# Autodesk Inventor assembly: Stewart-Platform-Innen
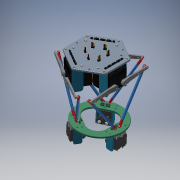
[picture p0: Inventor's stored thumbnail of the model, 180x180]
Saved by Autodesk Inventor 2018.2 (Build 222227000, 227)
## iProperties
Created: 2018-02-17
Part Number: Stewart-Platform-Innen
Material: Generisch
Document SubType Name: Assembly
Designer: JochenAlt
Author: JochenAlt
## Documents named in this file (11)
- D:\Projects\Donna\CAD\Stewart-Platform-Inside.iam
- D:\Projects\Donna\CAD\Servo-Holder.iam
- D:\Projects\Donna\CAD\Stewart-Platform-Base-Inside.ipt
- D:\Projects\Donna\CAD\Ball-Joint-Rod.iam
- D:\Projects\Donna\CAD\Servo-Arm-52mm-Ball-Joint.iam
- D:\Projects\Donna\CAD\Stewart-Plate-Inside.iam
- C:\Users\JochenAlt\Documents\Inventor\Content Center Files\R2018\de-DE\DIN 912\DIN 912 - M2 x 0,4 x 6 x 5.ipt
- C:\Users\JochenAlt\Documents\Inventor\Content Center Files\R2018\de-DE\AS 1112 (2)\AS 1112 - M2  Typ 5.ipt
- C:\Users\JochenAlt\Documents\Inventor\Content Center Files\R2018\de-DE\DIN 912\DIN 912 - M3 x 0,5 x 12 x 10,75.ipt
- C:\Users\JochenAlt\Documents\Inventor\Content Center Files\R2018\de-DE\DIN 912\DIN 912 - M3 x 0,5 x 10 x 8,75.ipt
- C:\Users\JochenAlt\Documents\Inventor\Content Center Files\R2018\de-DE\AS 1112 (2)\AS 1112 - M3  Typ 5.ipt
## Components (69 placed, 10 different names)
1. ServoHolder:1 [sub-assembly] — Passend:3, Passend:4, Passend:31, Passend:32, Passend:33, Passend:34, Passend:35, Passend:36, Passend:37, Passend:38, Passend:79, Passend:80, Passend:81, Passend:82, Passend:102, Passend:104, Passend:106, Passend:108, Passend:118, Passend:121, Passend:122, Passend:123, Passend:131, Passend:133
2. ServoHolder:2 [sub-assembly] — Passend:5, Passend:6, Einfügen:1, Einfügen:2, Einfügen:3, Einfügen:4, Passend:83, Passend:84, Passend:85, Passend:86, Passend:88, Passend:90, Passend:92, Passend:94, Passend:119, Passend:120, Passend:126, Passend:127, Passend:135
3. ServoHolder:3 [sub-assembly] — Passend:1, Passend:2, Passend:39, Passend:40, Passend:41, Passend:42, Passend:43, Passend:44, Passend:45, Passend:46, Passend:75, Passend:76, Passend:77, Passend:78, Passend:96, Einfügen:5, Passend:98, Passend:100, Passend:116, Passend:117, Passend:124, Passend:125, Passend:137, Passend:139
4. Stewart-Platform-Base:1 — Passend:1, Passend:2, Passend:3, Passend:4, Passend:5, Passend:6, Passend:48, Passend:50, Passend:52, Passend:54, Passend:56, Passend:58, Passend:60, Passend:62, Passend:64, Passend:66, Passend:68, Passend:70, Passend:71, Passend:72, Passend:73, Passend:74, Passend:128, Passend:129
5. Ball Joint Rod:1 [sub-assembly] — Passend:12, Passend:113
6. Ball Joint Rod:2 [sub-assembly] — Passend:9, Passend:115
7. Servo Lever ball joint:1 [sub-assembly] — Passend:12, Passend:121, Passend:122
8. Servo Lever ball joint:2 [sub-assembly] — Passend:9, Passend:118, Passend:123
9. Servo Lever ball joint:3 [sub-assembly] — Passend:18, Passend:117, Passend:125
10. Servo Lever ball joint:4 [sub-assembly] — Passend:17, Passend:116, Passend:124
11. Servo Lever ball joint:5 [sub-assembly] — Passend:24, Passend:119, Passend:127
12. Servo Lever ball joint:6 [sub-assembly] — Passend:23, Passend:120, Passend:126
13. Ball Joint Rod:3 [sub-assembly] — Passend:17, Passend:109
14. Ball Joint Rod:4 [sub-assembly] — Passend:18, Passend:110
15. Ball Joint Rod:5 [sub-assembly] — Passend:24, Passend:111
16. Ball Joint Rod:6 [sub-assembly] — Passend:23, Passend:114
17. DIN 912 - ersetzt durch DIN EN ISO 4762 M2 x 6:1 — Einfügen:1, Passend:53
18. DIN 912 - ersetzt durch DIN EN ISO 4762 M2 x 6:2 — Einfügen:2, Passend:47
19. DIN 912 - ersetzt durch DIN EN ISO 4762 M2 x 6:3 — Einfügen:3, Passend:49
20. DIN 912 - ersetzt durch DIN EN ISO 4762 M2 x 6:4 — Einfügen:4, Passend:51
21. DIN 912 - ersetzt durch DIN EN ISO 4762 M2 x 6:5 — Passend:31, Passend:32, Passend:67
22. DIN 912 - ersetzt durch DIN EN ISO 4762 M2 x 6:6 — Passend:33, Passend:34, Passend:63
23. DIN 912 - ersetzt durch DIN EN ISO 4762 M2 x 6:7 — Passend:35, Passend:36, Passend:65
24. DIN 912 - ersetzt durch DIN EN ISO 4762 M2 x 6:8 — Passend:37, Passend:38, Passend:69
25. DIN 912 - ersetzt durch DIN EN ISO 4762 M2 x 6:9 — Passend:39, Passend:40, Passend:55
26. DIN 912 - ersetzt durch DIN EN ISO 4762 M2 x 6:10 — Passend:41, Passend:42, Passend:57
27. DIN 912 - ersetzt durch DIN EN ISO 4762 M2 x 6:11 — Passend:43, Passend:44, Passend:59
28. DIN 912 - ersetzt durch DIN EN ISO 4762 M2 x 6:12 — Passend:45, Passend:46, Passend:61
29. AS 1112 (2) - Metrisch M2  Typ 5:1 — Passend:47, Passend:48
30. AS 1112 (2) - Metrisch M2  Typ 5:2 — Passend:49, Passend:50
31. AS 1112 (2) - Metrisch M2  Typ 5:3 — Passend:51, Passend:52
32. AS 1112 (2) - Metrisch M2  Typ 5:4 — Passend:53, Passend:54
33. AS 1112 (2) - Metrisch M2  Typ 5:5 — Passend:55, Passend:56
34. AS 1112 (2) - Metrisch M2  Typ 5:6 — Passend:57, Passend:58
35. AS 1112 (2) - Metrisch M2  Typ 5:7 — Passend:59, Passend:60
36. AS 1112 (2) - Metrisch M2  Typ 5:8 — Passend:61, Passend:62
37. AS 1112 (2) - Metrisch M2  Typ 5:9 — Passend:63, Passend:64
38. AS 1112 (2) - Metrisch M2  Typ 5:10 — Passend:65, Passend:66
39. AS 1112 (2) - Metrisch M2  Typ 5:11 — Passend:67, Passend:68
40. AS 1112 (2) - Metrisch M2  Typ 5:12 — Passend:69, Passend:70
41. DIN 912 - ersetzt durch DIN EN ISO 4762 M3 x 12:4 — Passend:73, Passend:74, Passend:138
42. DIN 912 - ersetzt durch DIN EN ISO 4762 M3 x 10:1 — Passend:75, Passend:76, Passend:97
43. DIN 912 - ersetzt durch DIN EN ISO 4762 M3 x 10:2 — Passend:77, Passend:78, Passend:99
44. DIN 912 - ersetzt durch DIN EN ISO 4762 M3 x 10:3 — Passend:79, Passend:80, Passend:101
45. DIN 912 - ersetzt durch DIN EN ISO 4762 M3 x 10:4 — Passend:81, Passend:82, Passend:107
46. DIN 912 - ersetzt durch DIN EN ISO 4762 M3 x 10:5 — Passend:83, Passend:84, Passend:89
47. DIN 912 - ersetzt durch DIN EN ISO 4762 M3 x 10:6 — Passend:85, Passend:86, Passend:93
48. AS 1112 (2) - Metrisch M3  Typ 5:1 — Passend:87, Passend:88
49. AS 1112 (2) - Metrisch M3  Typ 5:2 — Passend:89, Passend:90
50. AS 1112 (2) - Metrisch M3  Typ 5:3 — Passend:92
51. AS 1112 (2) - Metrisch M3  Typ 5:4 — Passend:93, Passend:94
52. AS 1112 (2) - Metrisch M3  Typ 5:5 — Passend:95, Passend:96
53. AS 1112 (2) - Metrisch M3  Typ 5:6 — Einfügen:5
54. AS 1112 (2) - Metrisch M3  Typ 5:7 — Passend:97, Passend:98
55. AS 1112 (2) - Metrisch M3  Typ 5:8 — Passend:99, Passend:100
56. AS 1112 (2) - Metrisch M3  Typ 5:9 — Passend:101, Passend:102
57. AS 1112 (2) - Metrisch M3  Typ 5:10 — Passend:104
58. AS 1112 (2) - Metrisch M3  Typ 5:11 — Passend:105, Passend:106
59. AS 1112 (2) - Metrisch M3  Typ 5:12 — Passend:107, Passend:108
60. Stewart-Plate:1 [sub-assembly] — Passend:109, Passend:110, Passend:111, Passend:113, Passend:114, Passend:115
61. DIN 912 - ersetzt durch DIN EN ISO 4762 M3 x 12:5 — Passend:128, Passend:129, Passend:130
62. AS 1112 (2) - Metrisch M3  Typ 5:13 — Passend:130, Passend:131
63. AS 1112 (2) - Metrisch M3  Typ 5:14 — Passend:132, Passend:133
64. AS 1112 (2) - Metrisch M3  Typ 5:15 — Passend:134, Passend:135
65. AS 1112 (2) - Metrisch M3  Typ 5:16 — Passend:136, Passend:137
66. AS 1112 (2) - Metrisch M3  Typ 5:17 — Passend:138, Passend:139
67. DIN 912 - ersetzt durch DIN EN ISO 4762 M3 x 12:1 — Passend:71, Passend:72, Passend:95, Passend:136
68. DIN 912 - ersetzt durch DIN EN ISO 4762 M3 x 12:2 — Passend:105, Passend:132
69. DIN 912 - ersetzt durch DIN EN ISO 4762 M3 x 12:3 — Passend:87, Passend:134
## Component patterns: (3 elements, first: DIN 912 - ersetzt durch DIN EN ISO 4762 M3 x 12:1)
## Relationships (123: Mate 118, Insert 5)
- Passend:1 [Mate]: ServoHolder:3 ↔ Stewart-Platform-Base:1
- Passend:2 [Mate]: ServoHolder:3 ↔ Stewart-Platform-Base:1
- Passend:3 [Mate]: ServoHolder:1 ↔ Stewart-Platform-Base:1
- Passend:4 [Mate]: ServoHolder:1 ↔ Stewart-Platform-Base:1
- Passend:5 [Mate]: ServoHolder:2 ↔ Stewart-Platform-Base:1
- Passend:6 [Mate]: ServoHolder:2 ↔ Stewart-Platform-Base:1
- Passend:9 [Mate]: Ball Joint Rod:2 ↔ Servo Lever ball joint:2
- Passend:12 [Mate]: Ball Joint Rod:1 ↔ Servo Lever ball joint:1
- Passend:17 [Mate]: Servo Lever ball joint:4 ↔ Ball Joint Rod:3
- Passend:18 [Mate]: Servo Lever ball joint:3 ↔ Ball Joint Rod:4
- Passend:23 [Mate]: Servo Lever ball joint:6 ↔ Ball Joint Rod:6
- Passend:24 [Mate]: Servo Lever ball joint:5 ↔ Ball Joint Rod:5
- Einfügen:1 [Insert]: ServoHolder:2 ↔ DIN 912 - ersetzt durch DIN EN ISO 4762 M2 x 6:1
- Einfügen:2 [Insert]: ServoHolder:2 ↔ DIN 912 - ersetzt durch DIN EN ISO 4762 M2 x 6:2
- Einfügen:3 [Insert]: ServoHolder:2 ↔ DIN 912 - ersetzt durch DIN EN ISO 4762 M2 x 6:3
- Einfügen:4 [Insert]: ServoHolder:2 ↔ DIN 912 - ersetzt durch DIN EN ISO 4762 M2 x 6:4
- Passend:31 [Mate]: ServoHolder:1 ↔ DIN 912 - ersetzt durch DIN EN ISO 4762 M2 x 6:5
- Passend:32 [Mate]: ServoHolder:1 ↔ DIN 912 - ersetzt durch DIN EN ISO 4762 M2 x 6:5
- Passend:33 [Mate]: ServoHolder:1 ↔ DIN 912 - ersetzt durch DIN EN ISO 4762 M2 x 6:6
- Passend:34 [Mate]: ServoHolder:1 ↔ DIN 912 - ersetzt durch DIN EN ISO 4762 M2 x 6:6
- Passend:35 [Mate]: ServoHolder:1 ↔ DIN 912 - ersetzt durch DIN EN ISO 4762 M2 x 6:7
- Passend:36 [Mate]: ServoHolder:1 ↔ DIN 912 - ersetzt durch DIN EN ISO 4762 M2 x 6:7
- Passend:37 [Mate]: ServoHolder:1 ↔ DIN 912 - ersetzt durch DIN EN ISO 4762 M2 x 6:8
- Passend:38 [Mate]: ServoHolder:1 ↔ DIN 912 - ersetzt durch DIN EN ISO 4762 M2 x 6:8
- Passend:39 [Mate]: ServoHolder:3 ↔ DIN 912 - ersetzt durch DIN EN ISO 4762 M2 x 6:9
- Passend:40 [Mate]: ServoHolder:3 ↔ DIN 912 - ersetzt durch DIN EN ISO 4762 M2 x 6:9
- Passend:41 [Mate]: ServoHolder:3 ↔ DIN 912 - ersetzt durch DIN EN ISO 4762 M2 x 6:10
- Passend:42 [Mate]: ServoHolder:3 ↔ DIN 912 - ersetzt durch DIN EN ISO 4762 M2 x 6:10
- Passend:43 [Mate]: ServoHolder:3 ↔ DIN 912 - ersetzt durch DIN EN ISO 4762 M2 x 6:11
- Passend:44 [Mate]: ServoHolder:3 ↔ DIN 912 - ersetzt durch DIN EN ISO 4762 M2 x 6:11
- Passend:45 [Mate]: ServoHolder:3 ↔ DIN 912 - ersetzt durch DIN EN ISO 4762 M2 x 6:12
- Passend:46 [Mate]: ServoHolder:3 ↔ DIN 912 - ersetzt durch DIN EN ISO 4762 M2 x 6:12
- Passend:47 [Mate]: DIN 912 - ersetzt durch DIN EN ISO 4762 M2 x 6:2 ↔ AS 1112 (2) - Metrisch M2  Typ 5:1
- Passend:48 [Mate]: Stewart-Platform-Base:1 ↔ AS 1112 (2) - Metrisch M2  Typ 5:1
- Passend:49 [Mate]: DIN 912 - ersetzt durch DIN EN ISO 4762 M2 x 6:3 ↔ AS 1112 (2) - Metrisch M2  Typ 5:2
- Passend:50 [Mate]: Stewart-Platform-Base:1 ↔ AS 1112 (2) - Metrisch M2  Typ 5:2
- Passend:51 [Mate]: DIN 912 - ersetzt durch DIN EN ISO 4762 M2 x 6:4 ↔ AS 1112 (2) - Metrisch M2  Typ 5:3
- Passend:52 [Mate]: Stewart-Platform-Base:1 ↔ AS 1112 (2) - Metrisch M2  Typ 5:3
- Passend:53 [Mate]: DIN 912 - ersetzt durch DIN EN ISO 4762 M2 x 6:1 ↔ AS 1112 (2) - Metrisch M2  Typ 5:4
- Passend:54 [Mate]: Stewart-Platform-Base:1 ↔ AS 1112 (2) - Metrisch M2  Typ 5:4
- Passend:55 [Mate]: DIN 912 - ersetzt durch DIN EN ISO 4762 M2 x 6:9 ↔ AS 1112 (2) - Metrisch M2  Typ 5:5
- Passend:56 [Mate]: Stewart-Platform-Base:1 ↔ AS 1112 (2) - Metrisch M2  Typ 5:5
- Passend:57 [Mate]: DIN 912 - ersetzt durch DIN EN ISO 4762 M2 x 6:10 ↔ AS 1112 (2) - Metrisch M2  Typ 5:6
- Passend:58 [Mate]: Stewart-Platform-Base:1 ↔ AS 1112 (2) - Metrisch M2  Typ 5:6
- Passend:59 [Mate]: DIN 912 - ersetzt durch DIN EN ISO 4762 M2 x 6:11 ↔ AS 1112 (2) - Metrisch M2  Typ 5:7
- Passend:60 [Mate]: Stewart-Platform-Base:1 ↔ AS 1112 (2) - Metrisch M2  Typ 5:7
- Passend:61 [Mate]: DIN 912 - ersetzt durch DIN EN ISO 4762 M2 x 6:12 ↔ AS 1112 (2) - Metrisch M2  Typ 5:8
- Passend:62 [Mate]: Stewart-Platform-Base:1 ↔ AS 1112 (2) - Metrisch M2  Typ 5:8
- Passend:63 [Mate]: DIN 912 - ersetzt durch DIN EN ISO 4762 M2 x 6:6 ↔ AS 1112 (2) - Metrisch M2  Typ 5:9
- Passend:64 [Mate]: Stewart-Platform-Base:1 ↔ AS 1112 (2) - Metrisch M2  Typ 5:9
- Passend:65 [Mate]: DIN 912 - ersetzt durch DIN EN ISO 4762 M2 x 6:7 ↔ AS 1112 (2) - Metrisch M2  Typ 5:10
- Passend:66 [Mate]: Stewart-Platform-Base:1 ↔ AS 1112 (2) - Metrisch M2  Typ 5:10
- Passend:67 [Mate]: DIN 912 - ersetzt durch DIN EN ISO 4762 M2 x 6:5 ↔ AS 1112 (2) - Metrisch M2  Typ 5:11
- Passend:68 [Mate]: Stewart-Platform-Base:1 ↔ AS 1112 (2) - Metrisch M2  Typ 5:11
- Passend:69 [Mate]: DIN 912 - ersetzt durch DIN EN ISO 4762 M2 x 6:8 ↔ AS 1112 (2) - Metrisch M2  Typ 5:12
- Passend:70 [Mate]: Stewart-Platform-Base:1 ↔ AS 1112 (2) - Metrisch M2  Typ 5:12
- Passend:71 [Mate]: Stewart-Platform-Base:1 ↔ DIN 912 - ersetzt durch DIN EN ISO 4762 M3 x 12:1
- Passend:72 [Mate]: Stewart-Platform-Base:1 ↔ DIN 912 - ersetzt durch DIN EN ISO 4762 M3 x 12:1
- Passend:73 [Mate]: Stewart-Platform-Base:1 ↔ DIN 912 - ersetzt durch DIN EN ISO 4762 M3 x 12:4
- Passend:74 [Mate]: Stewart-Platform-Base:1 ↔ DIN 912 - ersetzt durch DIN EN ISO 4762 M3 x 12:4
- Passend:75 [Mate]: ServoHolder:3 ↔ DIN 912 - ersetzt durch DIN EN ISO 4762 M3 x 10:1
- Passend:76 [Mate]: ServoHolder:3 ↔ DIN 912 - ersetzt durch DIN EN ISO 4762 M3 x 10:1
- Passend:77 [Mate]: ServoHolder:3 ↔ DIN 912 - ersetzt durch DIN EN ISO 4762 M3 x 10:2
- Passend:78 [Mate]: ServoHolder:3 ↔ DIN 912 - ersetzt durch DIN EN ISO 4762 M3 x 10:2
- Passend:79 [Mate]: ServoHolder:1 ↔ DIN 912 - ersetzt durch DIN EN ISO 4762 M3 x 10:3
- Passend:80 [Mate]: ServoHolder:1 ↔ DIN 912 - ersetzt durch DIN EN ISO 4762 M3 x 10:3
- Passend:81 [Mate]: ServoHolder:1 ↔ DIN 912 - ersetzt durch DIN EN ISO 4762 M3 x 10:4
- Passend:82 [Mate]: ServoHolder:1 ↔ DIN 912 - ersetzt durch DIN EN ISO 4762 M3 x 10:4
- Passend:83 [Mate]: ServoHolder:2 ↔ DIN 912 - ersetzt durch DIN EN ISO 4762 M3 x 10:5
- Passend:84 [Mate]: ServoHolder:2 ↔ DIN 912 - ersetzt durch DIN EN ISO 4762 M3 x 10:5
- Passend:85 [Mate]: ServoHolder:2 ↔ DIN 912 - ersetzt durch DIN EN ISO 4762 M3 x 10:6
- Passend:86 [Mate]: ServoHolder:2 ↔ DIN 912 - ersetzt durch DIN EN ISO 4762 M3 x 10:6
- Passend:87 [Mate]: AS 1112 (2) - Metrisch M3  Typ 5:1 ↔ DIN 912 - ersetzt durch DIN EN ISO 4762 M3 x 12:3
- Passend:88 [Mate]: ServoHolder:2 ↔ AS 1112 (2) - Metrisch M3  Typ 5:1
- Passend:89 [Mate]: DIN 912 - ersetzt durch DIN EN ISO 4762 M3 x 10:5 ↔ AS 1112 (2) - Metrisch M3  Typ 5:2
- Passend:90 [Mate]: ServoHolder:2 ↔ AS 1112 (2) - Metrisch M3  Typ 5:2
- Passend:92 [Mate]: ServoHolder:2 ↔ AS 1112 (2) - Metrisch M3  Typ 5:3
- Passend:93 [Mate]: DIN 912 - ersetzt durch DIN EN ISO 4762 M3 x 10:6 ↔ AS 1112 (2) - Metrisch M3  Typ 5:4
- Passend:94 [Mate]: ServoHolder:2 ↔ AS 1112 (2) - Metrisch M3  Typ 5:4
- Passend:95 [Mate]: AS 1112 (2) - Metrisch M3  Typ 5:5 ↔ DIN 912 - ersetzt durch DIN EN ISO 4762 M3 x 12:1
- Passend:96 [Mate]: ServoHolder:3 ↔ AS 1112 (2) - Metrisch M3  Typ 5:5
- Einfügen:5 [Insert]: ServoHolder:3 ↔ AS 1112 (2) - Metrisch M3  Typ 5:6
- Passend:97 [Mate]: DIN 912 - ersetzt durch DIN EN ISO 4762 M3 x 10:1 ↔ AS 1112 (2) - Metrisch M3  Typ 5:7
- Passend:98 [Mate]: ServoHolder:3 ↔ AS 1112 (2) - Metrisch M3  Typ 5:7
- Passend:99 [Mate]: DIN 912 - ersetzt durch DIN EN ISO 4762 M3 x 10:2 ↔ AS 1112 (2) - Metrisch M3  Typ 5:8
- Passend:100 [Mate]: ServoHolder:3 ↔ AS 1112 (2) - Metrisch M3  Typ 5:8
- Passend:101 [Mate]: DIN 912 - ersetzt durch DIN EN ISO 4762 M3 x 10:3 ↔ AS 1112 (2) - Metrisch M3  Typ 5:9
- Passend:102 [Mate]: ServoHolder:1 ↔ AS 1112 (2) - Metrisch M3  Typ 5:9
- Passend:104 [Mate]: ServoHolder:1 ↔ AS 1112 (2) - Metrisch M3  Typ 5:10
- Passend:105 [Mate]: AS 1112 (2) - Metrisch M3  Typ 5:11 ↔ DIN 912 - ersetzt durch DIN EN ISO 4762 M3 x 12:2
- Passend:106 [Mate]: ServoHolder:1 ↔ AS 1112 (2) - Metrisch M3  Typ 5:11
- Passend:107 [Mate]: DIN 912 - ersetzt durch DIN EN ISO 4762 M3 x 10:4 ↔ AS 1112 (2) - Metrisch M3  Typ 5:12
- Passend:108 [Mate]: ServoHolder:1 ↔ AS 1112 (2) - Metrisch M3  Typ 5:12
- Passend:109 [Mate]: Ball Joint Rod:3 ↔ Stewart-Plate:1
- Passend:110 [Mate]: Ball Joint Rod:4 ↔ Stewart-Plate:1
- Passend:111 [Mate]: Ball Joint Rod:5 ↔ Stewart-Plate:1
- Passend:113 [Mate]: Ball Joint Rod:1 ↔ Stewart-Plate:1
- Passend:114 [Mate]: Ball Joint Rod:6 ↔ Stewart-Plate:1
- Passend:115 [Mate]: Ball Joint Rod:2 ↔ Stewart-Plate:1
- Passend:116 [Mate]: ServoHolder:3 ↔ Servo Lever ball joint:4
- Passend:117 [Mate]: ServoHolder:3 ↔ Servo Lever ball joint:3
- Passend:118 [Mate]: ServoHolder:1 ↔ Servo Lever ball joint:2
- Passend:119 [Mate]: ServoHolder:2 ↔ Servo Lever ball joint:5
- Passend:120 [Mate]: ServoHolder:2 ↔ Servo Lever ball joint:6
- Passend:121 [Mate]: ServoHolder:1 ↔ Servo Lever ball joint:1
- Passend:122 [Mate]: ServoHolder:1 ↔ Servo Lever ball joint:1
- Passend:123 [Mate]: ServoHolder:1 ↔ Servo Lever ball joint:2
- Passend:124 [Mate]: ServoHolder:3 ↔ Servo Lever ball joint:4
- Passend:125 [Mate]: ServoHolder:3 ↔ Servo Lever ball joint:3
- Passend:126 [Mate]: ServoHolder:2 ↔ Servo Lever ball joint:6
- Passend:127 [Mate]: ServoHolder:2 ↔ Servo Lever ball joint:5
- Passend:128 [Mate]: Stewart-Platform-Base:1 ↔ DIN 912 - ersetzt durch DIN EN ISO 4762 M3 x 12:5
- Passend:129 [Mate]: Stewart-Platform-Base:1 ↔ DIN 912 - ersetzt durch DIN EN ISO 4762 M3 x 12:5
- Passend:130 [Mate]: DIN 912 - ersetzt durch DIN EN ISO 4762 M3 x 12:5 ↔ AS 1112 (2) - Metrisch M3  Typ 5:13
- Passend:131 [Mate]: ServoHolder:1 ↔ AS 1112 (2) - Metrisch M3  Typ 5:13
- Passend:132 [Mate]: AS 1112 (2) - Metrisch M3  Typ 5:14 ↔ DIN 912 - ersetzt durch DIN EN ISO 4762 M3 x 12:2
- Passend:133 [Mate]: ServoHolder:1 ↔ AS 1112 (2) - Metrisch M3  Typ 5:14
- Passend:134 [Mate]: AS 1112 (2) - Metrisch M3  Typ 5:15 ↔ DIN 912 - ersetzt durch DIN EN ISO 4762 M3 x 12:3
- Passend:135 [Mate]: ServoHolder:2 ↔ AS 1112 (2) - Metrisch M3  Typ 5:15
- Passend:136 [Mate]: AS 1112 (2) - Metrisch M3  Typ 5:16 ↔ DIN 912 - ersetzt durch DIN EN ISO 4762 M3 x 12:1
- Passend:137 [Mate]: ServoHolder:3 ↔ AS 1112 (2) - Metrisch M3  Typ 5:16
- Passend:138 [Mate]: DIN 912 - ersetzt durch DIN EN ISO 4762 M3 x 12:4 ↔ AS 1112 (2) - Metrisch M3  Typ 5:17
- Passend:139 [Mate]: ServoHolder:3 ↔ AS 1112 (2) - Metrisch M3  Typ 5:17
